# Autodesk Inventor assembly: PushRodSealAssembly0
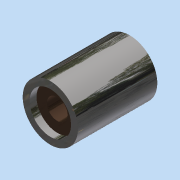
[picture p0: Inventor's stored thumbnail of the model, 180x180]
Saved by Autodesk Inventor 2017 (Build 210142000, 142)
## iProperties
Created: 2016-10-14
Part Number: PushRodSealAssembly0
Document SubType Name: Assembly
Designer: techn
Author: techn
## Documents named in this file (4)
- D:\OneDrive\Documents\Other Projects\Submarine\CAD\common\PushRodSeal\PushRodSealAssembly0.iam
- D:\OneDrive\Documents\Other Projects\Submarine\CAD\common\PushRodSeal\3mmBronzeBearings.ipt
- D:\OneDrive\Documents\Other Projects\Submarine\CAD\common\PushRodSeal\3mmXProfileORing.ipt
- D:\OneDrive\Documents\Other Projects\Submarine\CAD\common\PushRodSeal\6mmTubingSealHousing.ipt
## Components (4 placed, 3 different names)
1. 3mmBronzeBearings:1 — Mate:1, Flush:1
2. 3mmXProfileORing:1 — Mate:3, Mate:4
3. 6mmTubingSealHousing:1 — Mate:1, Mate:2, Mate:3, Flush:1, Flush:2
4. 3mmBronzeBearings:2 — Mate:2, Mate:4, Flush:2
## Relationships (6: Mate 4, Flush 2)
- Mate:1: 3mmBronzeBearings:1 ↔ 6mmTubingSealHousing:1
- Mate:2: 6mmTubingSealHousing:1 ↔ 3mmBronzeBearings:2
- Mate:3: 3mmXProfileORing:1 ↔ 6mmTubingSealHousing:1
- Flush:1 (1 mm): 3mmBronzeBearings:1 ↔ 6mmTubingSealHousing:1
- Mate:4 (0.0203 mm): 3mmXProfileORing:1 ↔ 3mmBronzeBearings:2
- Flush:2 (1 mm): 6mmTubingSealHousing:1 ↔ 3mmBronzeBearings:2
